# Autodesk Inventor assembly: Chest
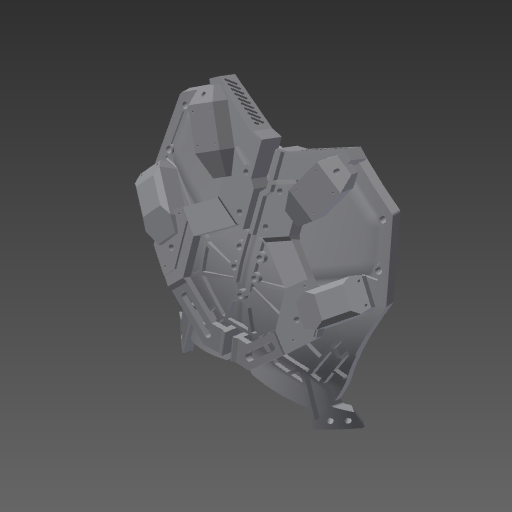
[picture p0: Inventor's stored thumbnail of the model, 512x512]
Saved by Autodesk Inventor 2020 (Build 240168000, 168)
## iProperties
Created: 2015-04-21
Part Number: Chest
Document SubType Name: Assembly
Designer: Val
Author: Val
## Documents named in this file (4)
- C:\Users\valer\Desktop\elysium-max-exoskeleton\src\Assemblies\Chest.iam
- C:\Users\valer\Desktop\elysium-max-exoskeleton\src\ChestBase.ipt
- C:\Users\valer\Desktop\elysium-max-exoskeleton\src\ChestPlateRight.ipt
- C:\Users\valer\Desktop\elysium-max-exoskeleton\src\ChestPlateLeft.ipt
## Components (3 placed, 3 different names)
1. ChestBase:1 — Mate:3
2. ChestPlateRight:1 — Flush:1, Flush:2, Mate:2, Mate:3
3. ChestPlateLeft:1 — Flush:1, Flush:2, Mate:2
## Relationships (4: Flush 2, Mate 2)
- Flush:1: ChestPlateRight:1 ↔ ChestPlateLeft:1
- Flush:2: ChestPlateRight:1 ↔ ChestPlateLeft:1
- Mate:2 (18 mm): ChestPlateRight:1 ↔ ChestPlateLeft:1
- Mate:3: ChestBase:1 ↔ ChestPlateRight:1
